# Autodesk Inventor assembly: Assembly_Lens_Thorlabs_Mount_KES400_Bluraylasermount
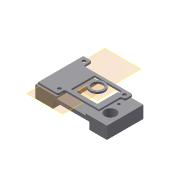
[picture p0: Inventor's stored thumbnail of the model, 180x180]
Saved by Autodesk Inventor 2019 (Build 230136000, 136)
## iProperties
Created: 2018-10-09
Part Number: Assembly_Lens_Thorlabs_Mount_KES400_Bluraylasermount
Document SubType Name: Assembly
Designer: diederichbenedict
Author: diederichbenedict
## Documents named in this file (3)
- C:\Users\diederichbenedict\Dropbox\Dokumente\Promotion\PROJECTS\STORMoChip\INVENTOR\Workspaces\Arbeitsbereich\10_Cube_Base\Assembly_Lens_Thorlabs_Mount_KES400_Bluraylasermount.iam
- C:\Users\diederichbenedict\Dropbox\Dokumente\Promotion\PROJECTS\STORMoChip\INVENTOR\Workspaces\Arbeitsbereich\10_Cube_Base\20_Adapter_Bluray_KES400_Lens_Thorlabs.ipt
- C:\Users\diederichbenedict\Dropbox\Dokumente\Promotion\PROJECTS\STORMoChip\INVENTOR\Workspaces\Arbeitsbereich\10_Cube_Base\00_KES400_Bluray_Lens.ipt
## Components (2 placed, 2 different names)
1. 00_KES400_Bluray_Lens:1 — Mate:1
2. 20_Adapter_Bluray_KES400_Lens_Thorlabs:1 — Mate:1
## Relationships (1: Mate 1)
- Mate:1: 00_KES400_Bluray_Lens:1 ↔ 20_Adapter_Bluray_KES400_Lens_Thorlabs:1
